# Autodesk Inventor assembly: Разъём с предохранителем и выключателем
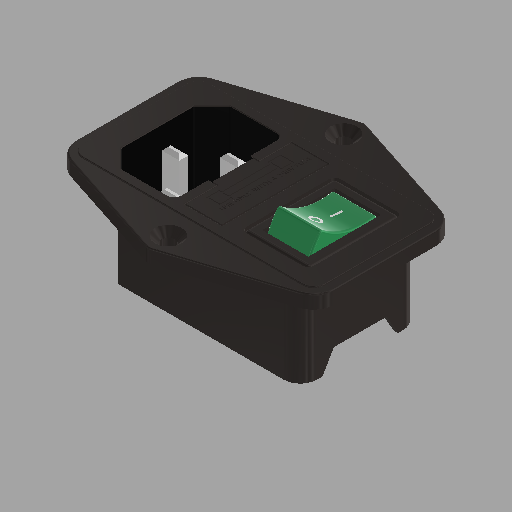
[picture p0: Inventor's stored thumbnail of the model, 512x512]
Saved by Autodesk Inventor 2023 (Build 270158000, 158)
## iProperties
Created: 2021-05-30
Part Number: Разъём с предохранителем и выключателем
Document SubType Name: Assembly
Designer: Mikhail
Author: Mikhail
## Documents named in this file (3)
- C:\Users\jan\Documents\Zeichenmaschine_neu\step Dateien\connector-with-switch-and-fuse-3.snapshot.1\baugruppe.iam
- C:\Users\jan\Documents\Zeichenmaschine_neu\step Dateien\connector-with-switch-and-fuse-3.snapshot.1\ARCOLECTRIC_H8600VB.ipt
- C:\Users\jan\Documents\Zeichenmaschine_neu\step Dateien\connector-with-switch-and-fuse-3.snapshot.1\part.ipt
## Components (2 placed, 2 different names)
1. ARCOLECTRIC_H8600VB:1 — Заподлицо:1, Заподлицо:2, Заподлицо:3
2. part:1 — Заподлицо:1, Заподлицо:2, Заподлицо:3
## Relationships (3: Flush 3)
- Заподлицо:1 [Flush]: ARCOLECTRIC_H8600VB:1 ↔ part:1
- Заподлицо:2 [Flush] (5 mm): ARCOLECTRIC_H8600VB:1 ↔ part:1
- Заподлицо:3 [Flush] (3.8 mm): ARCOLECTRIC_H8600VB:1 ↔ part:1
